# Autodesk Inventor assembly: Support
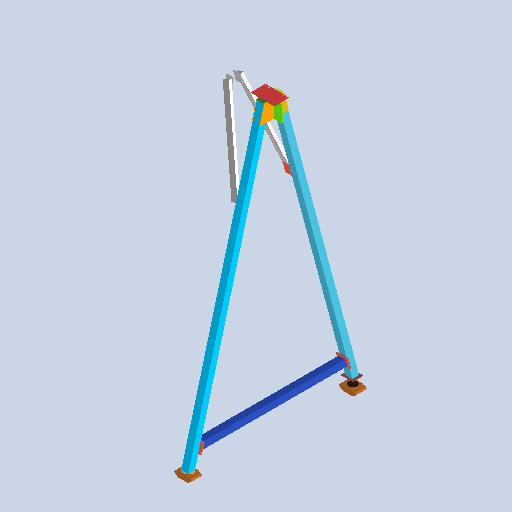
[picture p0: Inventor's stored thumbnail of the model, 512x512]
Saved by Autodesk Inventor 2025 (Build 290162010, 162A)
## iProperties
Created: 2024-06-18
Part Number: Support
Document SubType Name: Assembly
Designer: admin
Stock Number: Опора
Author: admin
## Documents named in this file (14)
- C:\Users\user\YandexDisk\домашниий пк\Inventor\Workshop\оборудование\Goat 2\Support.iam
- C:\Users\user\YandexDisk\домашниий пк\Inventor\Workshop\оборудование\Goat 2\Сrane plate 3.ipt
- C:\Users\user\YandexDisk\домашниий пк\Inventor\Workshop\оборудование\Goat 2\Stand.ipt
- C:\Users\user\YandexDisk\домашниий пк\Inventor\Workshop\оборудование\Goat 2\Сrane plate 4.ipt
- C:\Users\user\YandexDisk\домашниий пк\Inventor\Workshop\оборудование\Goat 2\Сrane plate 6.ipt
- C:\Users\user\YandexDisk\домашниий пк\Inventor\Workshop\оборудование\Goat 2\Сrane plate 2.ipt
- C:\Users\user\YandexDisk\домашниий пк\Inventor\Workshop\оборудование\Goat 2\Сrane plate 5.ipt
- C:\Users\user\YandexDisk\домашниий пк\Inventor\Workshop\оборудование\Goat 2\roller platform.ipt
- C:\Users\user\YandexDisk\домашниий пк\Inventor\Workshop\оборудование\Goat 2\foot.ipt
- C:\Users\user\YandexDisk\домашниий пк\Inventor\Workshop\оборудование\Goat 2\Crossbar.ipt
- C:\Users\user\YandexDisk\домашниий пк\Inventor\Workshop\оборудование\Goat 2\Сrane plate 1.ipt
- C:\Users\user\YandexDisk\домашниий пк\Inventor\Workshop\оборудование\Goat 2\Drawback 1.iam
- C:\Users\user\YandexDisk\домашниий пк\Inventor\Workshop\оборудование\Goat 2\Drawback 2.iam
- C:\Users\user\YandexDisk\домашниий пк\Inventor\Workshop\оборудование\Goat 2\leg 1\ASY leg1.iam
## Components (18 placed, 13 different names)
1. Сrane plate 3.ipt:1 — Mate:11, Mate:12, Mate:13, Flush:6, Flush:7
2. Stand.ipt:1 — Mate:9, Mate:10, Rigid:1
3. Сrane plate 4.ipt:1
4. Сrane plate 6.ipt:1 — Rigid:7
5. Сrane plate 4.ipt:2
6. Сrane plate 2.ipt:1 — Mate:11, Mate:12, Mate:13
7. Сrane plate 5.ipt:1 — Mate:9, Mate:10
8. roller platform.ipt:1 — Rigid:2, Mate:14
9. foot.ipt:1 — Rigid:1, Rigid:2
10. roller platform.ipt:2
11. Сrane plate 5.ipt:2
12. Сrane plate 6.ipt:3 — Rigid:7
13. Сrane plate 6.ipt:4 — Mate:41
14. Crossbar.ipt:1 — Mate:39, Mate:40, Mate:41
15. Сrane plate 1.ipt:1
16. Drawback 1.iam:1 [sub-assembly]
17. Drawback 2.iam:1 [sub-assembly]
18. ASY leg1:1 [sub-assembly]
## Relationships (40: Mate 23, Flush 9, WeldJoint 6, RevoluteJoint 2)
- [Mate]: Stand.ipt:1 ↔ Сrane plate 4.ipt:1
- [Mate]: Stand.ipt:1 ↔ Сrane plate 4.ipt:2
- [Flush]: Stand.ipt:1 ↔ Сrane plate 4.ipt:2
- [Flush]: Stand.ipt:1 ↔ Сrane plate 4.ipt:1
- [Flush]: Stand.ipt:1 ↔ Сrane plate 4.ipt:1
- [Flush]: Stand.ipt:1 ↔ Сrane plate 4.ipt:2
- [Flush]: Stand.ipt:1 ↔ Сrane plate 2.ipt:1
- [Mate]: Stand.ipt:1 ↔ Сrane plate 2.ipt:1
- [Mate]: Stand.ipt:1 ↔ Сrane plate 6.ipt:1
- [Mate]: Stand.ipt:1 ↔ Сrane plate 6.ipt:1
- [Mate]: Сrane plate 3.ipt:1 ↔ Сrane plate 4.ipt:2
- [Mate] (-200 mm): Stand.ipt:1 ↔ Сrane plate 6.ipt:1
- [Mate]: Stand.ipt:1 ↔ Сrane plate 5.ipt:1
- Mate:9 (-45 mm): Stand.ipt:1 ↔ Сrane plate 5.ipt:1
- Mate:10 (1271 mm): Stand.ipt:1 ↔ Сrane plate 5.ipt:1
- Mate:11: Сrane plate 3.ipt:1 ↔ Сrane plate 2.ipt:1
- Mate:12: Сrane plate 3.ipt:1 ↔ Сrane plate 2.ipt:1
- Mate:13: Сrane plate 3.ipt:1 ↔ Сrane plate 2.ipt:1
- Flush:6: Сrane plate 3.ipt:1
- Flush:7: Сrane plate 3.ipt:1
- Rigid:1 [WeldJoint]: Stand.ipt:1 ↔ foot.ipt:1
- Rigid:2 [WeldJoint]: roller platform.ipt:1 ↔ foot.ipt:1
- Mate:14: roller platform.ipt:1
- [RevoluteJoint]: Сrane plate 5.ipt:1 ↔ Drawback 1.iam:1
- [WeldJoint]: Сrane plate 3.ipt:1 ↔ ASY leg1:1
- [Flush] (60 mm): ASY leg1:1
- [Mate] (60 mm): ASY leg1:1
- [Mate]: Сrane plate 5.ipt:1 ↔ Drawback 1.iam:1
- [Mate]: ASY leg1:1
- [Mate]: Сrane plate 5.ipt:2 ↔ ASY leg1:1
- [Flush] (45 mm): Сrane plate 5.ipt:2 ↔ ASY leg1:1
- [Mate] (1271 mm): Сrane plate 5.ipt:2 ↔ ASY leg1:1
- [RevoluteJoint]: Сrane plate 5.ipt:2 ↔ Drawback 2.iam:1
- [Mate]: Сrane plate 5.ipt:2 ↔ Drawback 2.iam:1
- Rigid:7 [WeldJoint]: Сrane plate 6.ipt:1 ↔ Сrane plate 6.ipt:3
- [WeldJoint]: Сrane plate 6.ipt:4 ↔ ASY leg1:1
- Mate:39: Crossbar.ipt:1
- Mate:40: Crossbar.ipt:1
- Mate:41 (26.8 mm): Сrane plate 6.ipt:4 ↔ Crossbar.ipt:1
- [WeldJoint]: Сrane plate 1.ipt:1 ↔ ASY leg1:1
